# Autodesk Inventor assembly: Lg Motor
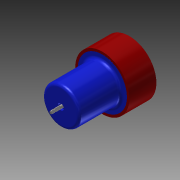
[picture p0: Inventor's stored thumbnail of the model, 180x180]
Saved by Autodesk Inventor 2013 (Build 170138000, 138)
## iProperties
Created: 2014-08-02
Part Number: Lg Motor
Document SubType Name: Assembly
Designer: Kyle
Author: Kyle
## Documents named in this file (4)
- C:\Users\Kyle\Documents\Autodesk\Inventor\Projects\ROV\Motor\Lg Motor.iam
- C:\Users\Kyle\Documents\Autodesk\Inventor\Projects\ROV\Motor\Lg Motor Bottom.ipt
- C:\Users\Kyle\Documents\Autodesk\Inventor\Projects\ROV\Motor\Lg Motor Top.ipt
- C:\Users\Kyle\Documents\Autodesk\Inventor\Projects\ROV\Motor\Lg Motor Shaft.ipt
## Components (3 placed, 3 different names)
1. Lg Motor Bottom:1 — Mate:1, Mate:2
2. Lg Motor Top:1 — Mate:1, Mate:2, Mate:3, Mate:4
3. Lg Motor Shaft:1 — Mate:3, Mate:4
## Relationships (4: Mate 4)
- Mate:1: Lg Motor Bottom:1 ↔ Lg Motor Top:1
- Mate:2: Lg Motor Bottom:1 ↔ Lg Motor Top:1
- Mate:3: Lg Motor Top:1 ↔ Lg Motor Shaft:1
- Mate:4: Lg Motor Top:1 ↔ Lg Motor Shaft:1
